# Autodesk Inventor assembly: 721112
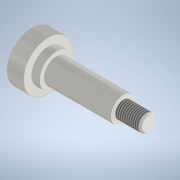
[picture p0: Inventor's stored thumbnail of the model, 180x180]
Saved by Autodesk Inventor 2022 (Build 260153000, 153)
## iProperties
Created: 2021-10-26
Part Number: 721112
Document SubType Name: Assembly
Designer: RaNSiD
Author: RaNSiD
## Documents named in this file (3)
- C:\Users\RaNSiD\Desktop\ВКР\Детали ЕСКД\721112.iam
- C:\Users\RaNSiD\Desktop\ВКР\Детали ЕСКД\Вал1.ipt
- C:\Users\RaNSiD\Desktop\ВКР\Детали ЕСКД\721112\Мастер проектирования\Цилиндрическое зубчатое зацепление1.iam
## Components (2 placed, 2 different names)
1. 721112 (Вал) — Совмещение:1
2. Цилиндрическое зубчатое зацепление:1 [sub-assembly] — Совмещение:1
## Relationships (1: Mate 1)
- Совмещение:1 [Mate]: 721112 (Вал) ↔ Цилиндрическое зубчатое зацепление:1
